# Autodesk Inventor assembly: main
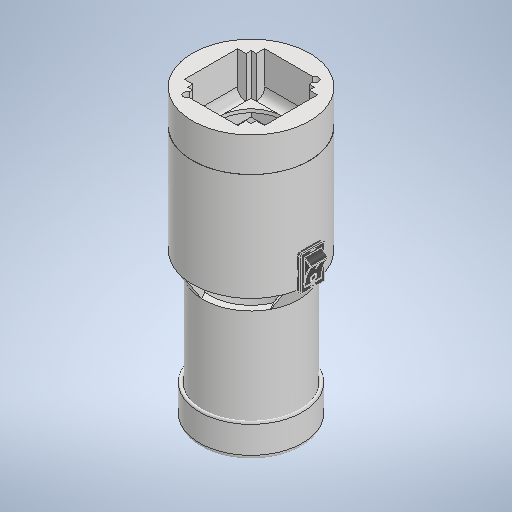
[picture p0: Inventor's stored thumbnail of the model, 512x512]
Saved by Autodesk Inventor 2025 (Build 290162000, 162)
## iProperties
Created: 2025-08-17
Part Number: main
Document SubType Name: Assembly
Designer: gavin
Author: gavin
## Documents named in this file (5)
- D:\Inventor\super flashlight v4\main.iam
- D:\Inventor\super flashlight v4\outercase.ipt
- D:\Inventor\super flashlight v4\super flash light v4 head.ipt
- D:\Inventor\super flashlight v4\super flash light v4.ipt
- D:\Inventor\super flashlight v4\Mini Rocker 4-Pin Switch\Mini Rocker 4-Pin Switch.ipt
## Components (4 placed, 4 different names)
1. outercase:1 — 剛性:1, 剛性:2, 貼合:1, 貼合:2, 相切:1
2. super flash light v4 head:1 — 剛性:2
3. super flash light v4:1 — 剛性:1
4. Mini Rocker 4-Pin Switch:1 — 貼合:1, 貼合:2, 相切:1
## Relationships (5: WeldJoint 2, Mate 2, Tangent 1)
- 剛性:1 [WeldJoint]: outercase:1 ↔ super flash light v4:1
- 剛性:2 [WeldJoint]: outercase:1 ↔ super flash light v4 head:1
- 貼合:1 [Mate]: outercase:1 ↔ Mini Rocker 4-Pin Switch:1
- 貼合:2 [Mate]: outercase:1 ↔ Mini Rocker 4-Pin Switch:1
- 相切:1 [Tangent]: outercase:1 ↔ Mini Rocker 4-Pin Switch:1
